# Autodesk Inventor assembly: ENSAMBLE BOMBA
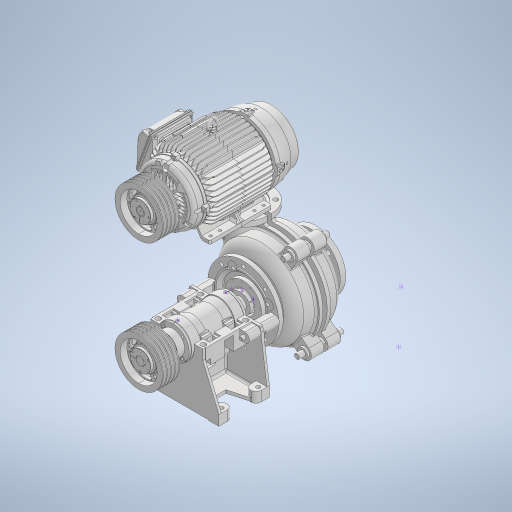
[picture p0: Inventor's stored thumbnail of the model, 512x512]
Saved by Autodesk Inventor 2024.1 (Build 281209000, 209)
## iProperties
Created: 2025-06-24
Part Number: ENSAMBLE BOMBA
Document SubType Name: Assembly
Designer: User
Author: User
## Documents named in this file (6)
- C:\Users\User\OneDrive\Documents\POLEAS\ENSAMBLE BOMBA.iam
- C:\Users\User\OneDrive\Documents\POLEAS\6209K324_Quick-Disconnect Bushing-Bore V-Belt Pulley.iam
- C:\Users\User\OneDrive\Documents\POLEAS\phf_sk-32mm.ipt
- C:\Users\User\OneDrive\Documents\POLEAS\MOTOR ELECTRICO WEG 75 HP\07568453.iam
- C:\Users\User\OneDrive\Documents\POLEAS\WARMAN 4X3 SOPORTE\WARMAN 4_3.iam
- C:\Users\User\OneDrive\Documents\POLEAS\phf_sk-42mm.ipt
## Components (6 placed, 5 different names)
1. 6209K324_Quick-Disconnect Bushing-Bore V-Belt Pulley:1 [sub-assembly] — Flush:1, Flush:2, Flush:3, Mate:1, Mate:2, Flush:10
2. phf_sk-32mm:1 — Mate:1, Mate:2, Flush:7, Flush:11
3. 07568453:1 [sub-assembly] — Flush:4, Flush:5, Flush:6, Flush:7, Mate:3, Flush:9
4. WARMAN 4_3:1 [sub-assembly] — Mate:3, Flush:8, Flush:9, Mate:4, Mate:5, Angle:1
5. phf_sk-42mm:1 — Mate:5, Angle:1, Mate:6, Flush:11
6. 6209K324_Quick-Disconnect Bushing-Bore V-Belt Pulley:2 [sub-assembly] — Mate:4, Flush:10, Mate:6
## Relationships (18: Flush 11, Mate 6, Angle 1)
- Flush:1: 6209K324_Quick-Disconnect Bushing-Bore V-Belt Pulley:1
- Flush:2: 6209K324_Quick-Disconnect Bushing-Bore V-Belt Pulley:1
- Flush:3 (-52 mm): 6209K324_Quick-Disconnect Bushing-Bore V-Belt Pulley:1
- Mate:1: 6209K324_Quick-Disconnect Bushing-Bore V-Belt Pulley:1 ↔ phf_sk-32mm:1
- Mate:2: 6209K324_Quick-Disconnect Bushing-Bore V-Belt Pulley:1 ↔ phf_sk-32mm:1
- Flush:4: 07568453:1
- Flush:5: 07568453:1
- Flush:6 (-200 mm): 07568453:1
- Flush:7: phf_sk-32mm:1 ↔ 07568453:1
- Mate:3 (200 mm): 07568453:1 ↔ WARMAN 4_3:1
- Flush:8: WARMAN 4_3:1
- Flush:9: 07568453:1 ↔ WARMAN 4_3:1
- Mate:4: WARMAN 4_3:1 ↔ 6209K324_Quick-Disconnect Bushing-Bore V-Belt Pulley:2
- Flush:10: 6209K324_Quick-Disconnect Bushing-Bore V-Belt Pulley:1 ↔ 6209K324_Quick-Disconnect Bushing-Bore V-Belt Pulley:2
- Mate:5: WARMAN 4_3:1 ↔ phf_sk-42mm:1
- Angle:1 (0 deg): WARMAN 4_3:1 ↔ phf_sk-42mm:1
- Mate:6: phf_sk-42mm:1 ↔ 6209K324_Quick-Disconnect Bushing-Bore V-Belt Pulley:2
- Flush:11: phf_sk-32mm:1 ↔ phf_sk-42mm:1
